# Autodesk Inventor assembly: Tank
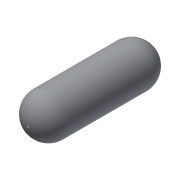
[picture p0: Inventor's stored thumbnail of the model, 180x180]
Saved by Autodesk Inventor 2015 (Build 190159000, 159)
## iProperties
Created: 2015-12-04
Part Number: Tank
Document SubType Name: Assembly
Designer: kbutz
Author: kbutz
## Documents named in this file (3)
- C:\Users\kbutz\Desktop\Model Shit\Tank.iam
- C:\Users\kbutz\Desktop\Model Shit\Cap.ipt
- C:\Users\kbutz\Desktop\Model Shit\tank.ipt
## Components (3 placed, 2 different names)
1. Cap:1 — Mate:1, Mate:2
2. tank:1 — Mate:1, Mate:2, Mate:3, Mate:4
3. Cap:2 — Mate:3, Mate:4
## Relationships (4: Mate 4)
- Mate:1: Cap:1 ↔ tank:1
- Mate:2: Cap:1 ↔ tank:1
- Mate:3: tank:1 ↔ Cap:2
- Mate:4: tank:1 ↔ Cap:2
